# Autodesk Inventor assembly: Case assembly
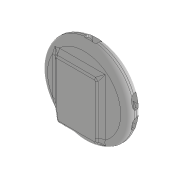
[picture p0: Inventor's stored thumbnail of the model, 180x180]
Saved by Autodesk Inventor 2020 (Build 240168000, 168)
## iProperties
Created: 2022-04-09
Part Number: Case assembly
Document SubType Name: Assembly
Designer: ferrerx
Author: ferrerx
## Documents named in this file (3)
- C:\Users\ferrerx\Documents\GitHub\Wireless_EMG\Design files\Case assembly.iam
- C:\Users\ferrerx\Documents\GitHub\Wireless_EMG\Design files\Case top.ipt
- C:\Users\ferrerx\Documents\GitHub\Wireless_EMG\Design files\Case bottom V2.ipt
## Components (2 placed, 2 different names)
1. Case top:1 — Mate:1, Mate:2, Mate:3
2. Case bottom V2:1 — Mate:1, Mate:2, Mate:3
## Relationships (3: Mate 3)
- Mate:1: Case top:1 ↔ Case bottom V2:1
- Mate:2: Case top:1 ↔ Case bottom V2:1
- Mate:3 (1.6 mm): Case top:1 ↔ Case bottom V2:1
